# Autodesk Inventor assembly: BoltWasher3x24
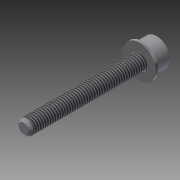
[picture p0: Inventor's stored thumbnail of the model, 180x180]
Saved by Autodesk Inventor 2015 SP1 (Build 190203100, 203)
## iProperties
Category: Hardware
Created: 2015-01-27
Part Number: BoltWasher3x24
Document SubType Name: Assembly
Designer: Jack
Vendor: Misumi
Mass: 0.338993 g
Surface Area: 4.09761 cm^2
Volume: 0.242655 cm^3
Density: 1.39701 g/cm^3
Author: Jack
Title: Bolt + Washer 3x24
## Documents named in this file (3)
- C:\Users\Jack\ownCloud\Projects\CrossBot\InventorModel\Hardware\BoltWashers\BoltWasher3\BoltWasher3x24.iam
- C:\Users\Jack\ownCloud\Projects\CrossBot\InventorModel\Hardware\Wahsers\M3Washer.ipt
- C:\Users\Jack\ownCloud\Projects\CrossBot\InventorModel\Hardware\Bolts\SHCS\SHCS3\SHCS3x24.ipt
## Components (2 placed, 2 different names)
1. M3Washer:1 — Mate:1, Mate:2
2. SHCS3x24:1 — Mate:1, Mate:2
## Relationships (2: Mate 2)
- Mate:1: M3Washer:1 ↔ SHCS3x24:1
- Mate:2: M3Washer:1 ↔ SHCS3x24:1
